# Autodesk Inventor assembly: presentation
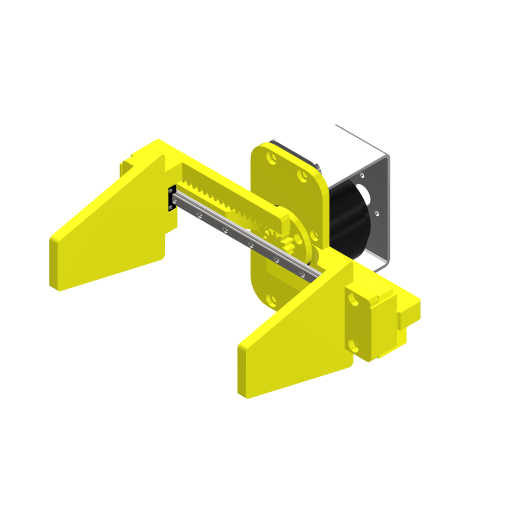
[picture p0: Inventor's stored thumbnail of the model, 512x512]
Saved by Autodesk Inventor 2023 (Build 270158000, 158)
## iProperties
Created: 2024-12-17
Part Number: presentation
Catalog Web Link: www.cadenas.de
Description: SSEB, SSEB-MX, SSE2B, SSE2B-MX, RSEB, RSE2B-Miniature Linear Guides Standard Blocks/Light Preload High Grade-L Selectable Type
Vendor: MISUMI
Document SubType Name: Assembly
Designer: psAdmin
Manufacturer: MISUMI
Mass: 135.965 g
Surface Area: 614.146 cm^2
Volume: 83.3375 cm^3
Density: 1.63149 g/cm^3
Category: PARTsolutions
Company: MISUMI
PSOL_IDENT_0: {$CADENAS_DATA/23d-libs/misumi/metric/06_linear_guides/re2b_asmtab.prj},256 {VTYP=3D},{STYP=ASSTAB},
PSOL_IDENT_1: {NB=SSE2B6-145},{LINA=SSE2B6-145},{NN=SSEB, SSEB-MX, SSE2B, SSE2B-MX, RSEB, RSE2B},{DATE=04.04.2024
PSOL_IDENT_2: 07:12:35},{GEOMDATE=07.03.2024 00:33:43},{VERSION=},{LINEID=60},{WBVAR=ST,MAT,MX,NOB,GREASE,LS,ALT1,
PSOL_IDENT_3: ALT2,ALT3,ALT4},{WBNUMERIC=LS}  {NB=SSE2B6-145},{LINA=SSE2B6-145},{KT=DUMMY},{PN=SSE2B6-145},{RT=B},
PSOL_IDENT_4: {TYPE=SSE2B},{ST=S},{MAT=S},{MX=},{MXALG= '','w/o MX(Lubrication unit)' },{NOB=2},{H=6},{GREASE=},{G
PSOL_IDENT_5: REASEALG='','Normal', 'L'  , 'L Type Greased ', 'G', 'G Type Greased', 'Y', 'Y Type Greased', 'H', '
PSOL_IDENT_6: H Type Greased'},{LT=Selectable},{LS=145},{HARD=56HRC~},{W=12},{L1=17.4},{B=8},{C=0},{SLL=M2x1.5},{L
PSOL_IDENT_7: 2=9.7},{K=4.5},{CBB=0.3},{W1=5},{W2=3.5},{H1=4.0},{CAA=0.3},{DD1DD2HH=2.4x3.5x1},{F=15},{G=5.0},{ALT
PSOL_IDENT_8: 1=},{ALT1ALG= '', 'w/o MC (Tapped Holes)' },{MC=M2.6},{ALT2=},{ALT2L=0.0},{ALT2N=0},{M=10},{LL=},{L0=
PSOL_IDENT_9: 70,85,100,115,130,145},{REC1=   '','Not applicable'    },{ST1='S', 'w/o Surface Treatment'},{MAT2='S'
PSOL_IDENT_10: ,'Stainless Steel'},{ALT3=},{ALT3ALG= '' , 'w/o WC (Pair of Rails)' , '-WC' , 'with WC (Set Pair of
PSOL_IDENT_11: Rails)' },{ALT4=},{ALT4ALG= '','N/A' },{PPATH=seb_series/seb_asmtpl.prj}
NB: SSE2B6-145
NN: SSEB, SSEB-MX, SSE2B, SSE2B-MX, RSEB, RSE2B
NT: Miniature Linear Guides Standard Blocks/Light Preload High Grade-L Selectable Type
NBSYN: $PN.
LINA: SSE2B6-145
CATALOG: Misumi
PN: SSE2B6-145
ST: w/o Surface Treatment
MAT: Stainless Steel
MX: w/o MX(Lubrication unit)
NOB: 2
H: 6
GREASE: Normal
LS: 145
W: 12
L1: 17.4
B: 8
C: 0
SLL: M2x1.5
L2: 9.7
K: 4.5
CBB: 0.3
W1: 5
W2: 3.5
H1: 4
CAA: 0.3
DD1DD2HH: 2.4x3.5x1
F: 15
G: 5
ALT1: w/o MC (Tapped Holes)
ALT2: Not applicable
ALT3: w/o WC (Pair of Rails)
ALT4: N/A
SUPPLIER: MISUMI
ARTICLENO: SSE2B6-145
BOMINFO: SSE2B6-145
CREATOR: CADENAS GmbH
Title: SSE2B6-145
Author: Cadenas PARTsolutions
Comments: Miniature Linear Guides Standard Blocks/Light Preload High Grade-L Selectable Type
## Documents named in this file (9)
- D:\GitHub\inventor\syu-si\OfficeRobot\Hand\presentation.iam
- D:\GitHub\inventor\syu-si\OfficeRobot\ReadyMade\linear_guide\SSE2B6-145\SSE2B6-145_r.ipt
- D:\GitHub\inventor\syu-si\OfficeRobot\ReadyMade\linear_guide\SSE2B6-145\SSEB6_b.ipt
- D:\GitHub\inventor\syu-si\OfficeRobot\Hand\linear-gear.ipt
- D:\GitHub\inventor\syu-si\OfficeRobot\Hand\fix-guide-motor.ipt
- D:\GitHub\inventor\syu-si\OfficeRobot\Hand\hand-gear.ipt
- D:\GitHub\inventor\syu-si\OfficeRobot\ReadyMade\Steadywin\GIM3505-8_with-driver.ipt
- D:\GitHub\inventor\syu-si\OfficeRobot\Hand\hand_box2.ipt
- D:\GitHub\inventor\syu-si\OfficeRobot\Hand\nail.ipt
## Components (11 placed, 8 different names)
1. hand_box2:1 — フラッシュ:2
2. GIM3505-8_with-driver:1
3. 平歯車1:1 — 角度:4
4. fix-guide-motor:1 — メイト:17, メイト:18
5. linear-gear:1 — 挿入:66, 角度:4, メイト:18
6. linear-gear:2 — 挿入:67, メイト:17
7. SSE2B6-145_r:1
8. SSEB6_b:1 — 挿入:66, 角度:5
9. SSEB6_b:2 — 挿入:67, 角度:3
10. nail:2 — 角度:5, フラッシュ:1
11. nail:3 — 角度:3, フラッシュ:3
## Relationships (19: Insert 7, Angle 5, Mate 4, Flush 3)
- [Insert]: GIM3505-8_with-driver:1 ↔ 平歯車1:1
- [Insert]: GIM3505-8_with-driver:1 ↔ fix-guide-motor:1
- [Insert]: GIM3505-8_with-driver:1 ↔ fix-guide-motor:1
- [Insert]: hand_box2:1 ↔ fix-guide-motor:1
- [Insert]: hand_box2:1 ↔ fix-guide-motor:1
- [Mate]: SSE2B6-145_r:1 ↔ SSEB6_b:1
- [Angle] (0 deg): SSE2B6-145_r:1 ↔ SSEB6_b:1
- [Mate]: SSE2B6-145_r:1 ↔ SSEB6_b:2
- [Angle] (0 deg): SSE2B6-145_r:1 ↔ SSEB6_b:2
- 挿入:66 [Insert]: linear-gear:1 ↔ SSEB6_b:1
- 挿入:67 [Insert]: linear-gear:2 ↔ SSEB6_b:2
- 角度:3 [Angle] (0 deg): SSEB6_b:2 ↔ nail:3
- 角度:4 [Angle] (0 deg): 平歯車1:1 ↔ linear-gear:1
- 角度:5 [Angle] (0 deg): SSEB6_b:1 ↔ nail:2
- フラッシュ:1 [Flush] (32 mm): nail:2
- メイト:17 [Mate]: fix-guide-motor:1 ↔ linear-gear:2
- メイト:18 [Mate]: fix-guide-motor:1 ↔ linear-gear:1
- フラッシュ:2 [Flush] (28.5 mm): hand_box2:1
- フラッシュ:3 [Flush] (57.5 mm): nail:3
